# Autodesk Inventor assembly: Flywheel Axle Assembly v11
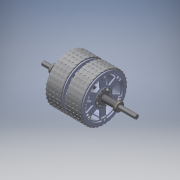
[picture p0: Inventor's stored thumbnail of the model, 180x180]
Saved by Autodesk Inventor 2018 (Build 220112000, 112)
## iProperties
Created: 2020-01-29
Part Number: Flywheel Axle Assembly v11
Document SubType Name: Assembly
Designer: s-2512711
Author: s-2512711
## Documents named in this file (10)
- \\studenthome\students\S-2512711\GitHub\2020CAD\New Gabriel Shooter\ACTUAL ASSEMBLY FILES\Flywheel Axle Assembly v11.iam
- \\studenthome\students\S-2512711\GitHub\2020CAD\New Gabriel Shooter\ACTUAL ASSEMBLY FILES\am-2986 FR8ZZ Hex Bearing v1.ipt
- \\studenthome\students\S-2512711\GitHub\2020CAD\New Gabriel Shooter\ACTUAL ASSEMBLY FILES\6_Traction_Tire_mounted_on_6_Traction_Wheel v1.iam
- \\studenthome\students\S-2512711\GitHub\2020CAD\New Gabriel Shooter\ACTUAL ASSEMBLY FILES\6_Traction_Tire_mounted_on_6_Traction_Wheel v1_1.iam
- \\studenthome\students\S-2512711\GitHub\2020CAD\New Gabriel Shooter\ACTUAL ASSEMBLY FILES\1_2_Hex_Bore_Aluminum_VersaHub_217-2592 v1.ipt
- \\studenthome\students\S-2512711\GitHub\2020CAD\New Gabriel Shooter\ACTUAL ASSEMBLY FILES\1_2_Acetal_Spacer_-_1_2_Hex_217-3261 v1.ipt
- \\studenthome\students\S-2512711\GitHub\2020CAD\New Gabriel Shooter\ACTUAL ASSEMBLY FILES\1_16_Acetal_Spacer_-_1_2_Hex_217-3257 v1.ipt
- \\studenthome\students\S-2512711\GitHub\2020CAD\New Gabriel Shooter\ACTUAL ASSEMBLY FILES\1_Acetal_Spacer_-_1_2_Hex_217-3263 v1.ipt
- \\studenthome\students\S-2512711\GitHub\2020CAD\New Gabriel Shooter\ACTUAL ASSEMBLY FILES\1_4_Acetal_Spacer_-_1_2_Hex_217-3259 v1.ipt
- \\studenthome\students\S-2512711\GitHub\2020CAD\New Gabriel Shooter\ACTUAL ASSEMBLY FILES\Flywheel Axle Assembly v11.ipt
## Components (18 placed, 8 different names)
1. am-2986 FR8ZZ Hex Bearing v1:1 — Mate:1, Mate:2, Flush:1
2. am-2986 FR8ZZ Hex Bearing v1:2 — Mate:30, Mate:31, Flush:8
3. 6_Traction_Tire_mounted_on_6_Traction_Wheel v1:1 [sub-assembly] — Mate:13, Mate:14, Mate:19, Mate:20
4. 6_Traction_Tire_mounted_on_6_Traction_Wheel v1:2 [sub-assembly] — Mate:24, Mate:25, Mate:26, Mate:29
5. 1_2_Hex_Bore_Aluminum_VersaHub_217-2592 v1:1 — Mate:11, Mate:12, Flush:6, Mate:13, Mate:14
6. 1_2_Hex_Bore_Aluminum_VersaHub_217-2592 v1:2 — Mate:17, Mate:18, Mate:19, Mate:20, Mate:23
7. 1_2_Hex_Bore_Aluminum_VersaHub_217-2592 v1:3 — Mate:15, Mate:16, Flush:7, Mate:24, Mate:25, Mate:26
8. 1_2_Hex_Bore_Aluminum_VersaHub_217-2592 v1:4 — Mate:27, Mate:28, Mate:29
9. 1_2_Acetal_Spacer_-_1_2_Hex_217-3261 v1:1 — Mate:21, Mate:22, Mate:23
10. 1_2_Acetal_Spacer_-_1_2_Hex_217-3261 v1:2 — Mate:7, Mate:8, Flush:4
11. 1_2_Acetal_Spacer_-_1_2_Hex_217-3261 v1:3 — Mate:36, Mate:37, Flush:11
12. 1_16_Acetal_Spacer_-_1_2_Hex_217-3257 v1:1 — Mate:32, Mate:33, Flush:9
13. 1_16_Acetal_Spacer_-_1_2_Hex_217-3257 v1:2 — Mate:3, Mate:4, Flush:2
14. 1_Acetal_Spacer_-_1_2_Hex_217-3263 v1:1 — Mate:38, Mate:39, Flush:12
15. 1_Acetal_Spacer_-_1_2_Hex_217-3263 v1:2 — Mate:9, Mate:10, Flush:5
16. 1_4_Acetal_Spacer_-_1_2_Hex_217-3259 v1:1 — Mate:5, Mate:6, Flush:3
17. 1_4_Acetal_Spacer_-_1_2_Hex_217-3259 v1:2 — Mate:34, Mate:35, Flush:10
18. Flywheel Axle Assembly v11 — Mate:1, Mate:2, Flush:1, Mate:3, Mate:4, Flush:2, Mate:5, Mate:6, Flush:3, Mate:7, Mate:8, Flush:4, Mate:9, Mate:10, Flush:5, Mate:11, Mate:12, Flush:6, Mate:15, Mate:16, Flush:7, Mate:17, Mate:18, Mate:21, Mate:22, Mate:27, Mate:28, Mate:30, Mate:31, Flush:8, Mate:32, Mate:33, Flush:9, Mate:34, Mate:35, Flush:10, Mate:36, Mate:37, Flush:11, Mate:38, Mate:39, Flush:12
## Relationships (51: Mate 39, Flush 12)
- Mate:1: am-2986 FR8ZZ Hex Bearing v1:1 ↔ Flywheel Axle Assembly v11
- Mate:2: am-2986 FR8ZZ Hex Bearing v1:1 ↔ Flywheel Axle Assembly v11
- Flush:1 (31.75 mm): am-2986 FR8ZZ Hex Bearing v1:1 ↔ Flywheel Axle Assembly v11
- Mate:3: 1_16_Acetal_Spacer_-_1_2_Hex_217-3257 v1:2 ↔ Flywheel Axle Assembly v11
- Mate:4: 1_16_Acetal_Spacer_-_1_2_Hex_217-3257 v1:2 ↔ Flywheel Axle Assembly v11
- Flush:2 (39.6875 mm): 1_16_Acetal_Spacer_-_1_2_Hex_217-3257 v1:2 ↔ Flywheel Axle Assembly v11
- Mate:5: 1_4_Acetal_Spacer_-_1_2_Hex_217-3259 v1:1 ↔ Flywheel Axle Assembly v11
- Mate:6: 1_4_Acetal_Spacer_-_1_2_Hex_217-3259 v1:1 ↔ Flywheel Axle Assembly v11
- Flush:3 (41.275 mm): 1_4_Acetal_Spacer_-_1_2_Hex_217-3259 v1:1 ↔ Flywheel Axle Assembly v11
- Mate:7: 1_2_Acetal_Spacer_-_1_2_Hex_217-3261 v1:2 ↔ Flywheel Axle Assembly v11
- Mate:8: 1_2_Acetal_Spacer_-_1_2_Hex_217-3261 v1:2 ↔ Flywheel Axle Assembly v11
- Flush:4 (47.625 mm): 1_2_Acetal_Spacer_-_1_2_Hex_217-3261 v1:2 ↔ Flywheel Axle Assembly v11
- Mate:9: 1_Acetal_Spacer_-_1_2_Hex_217-3263 v1:2 ↔ Flywheel Axle Assembly v11
- Mate:10: 1_Acetal_Spacer_-_1_2_Hex_217-3263 v1:2 ↔ Flywheel Axle Assembly v11
- Flush:5 (60.325 mm): 1_Acetal_Spacer_-_1_2_Hex_217-3263 v1:2 ↔ Flywheel Axle Assembly v11
- Mate:11: 1_2_Hex_Bore_Aluminum_VersaHub_217-2592 v1:1 ↔ Flywheel Axle Assembly v11
- Mate:12: 1_2_Hex_Bore_Aluminum_VersaHub_217-2592 v1:1 ↔ Flywheel Axle Assembly v11
- Flush:6 (85.725 mm): 1_2_Hex_Bore_Aluminum_VersaHub_217-2592 v1:1 ↔ Flywheel Axle Assembly v11
- Mate:13: 6_Traction_Tire_mounted_on_6_Traction_Wheel v1:1 ↔ 1_2_Hex_Bore_Aluminum_VersaHub_217-2592 v1:1
- Mate:14: 6_Traction_Tire_mounted_on_6_Traction_Wheel v1:1 ↔ 1_2_Hex_Bore_Aluminum_VersaHub_217-2592 v1:1
- Mate:15: 1_2_Hex_Bore_Aluminum_VersaHub_217-2592 v1:3 ↔ Flywheel Axle Assembly v11
- Mate:16: 1_2_Hex_Bore_Aluminum_VersaHub_217-2592 v1:3 ↔ Flywheel Axle Assembly v11
- Flush:7 (152.4 mm): 1_2_Hex_Bore_Aluminum_VersaHub_217-2592 v1:3 ↔ Flywheel Axle Assembly v11
- Mate:17: 1_2_Hex_Bore_Aluminum_VersaHub_217-2592 v1:2 ↔ Flywheel Axle Assembly v11
- Mate:18: 1_2_Hex_Bore_Aluminum_VersaHub_217-2592 v1:2 ↔ Flywheel Axle Assembly v11
- Mate:19: 6_Traction_Tire_mounted_on_6_Traction_Wheel v1:1 ↔ 1_2_Hex_Bore_Aluminum_VersaHub_217-2592 v1:2
- Mate:20: 6_Traction_Tire_mounted_on_6_Traction_Wheel v1:1 ↔ 1_2_Hex_Bore_Aluminum_VersaHub_217-2592 v1:2
- Mate:21: 1_2_Acetal_Spacer_-_1_2_Hex_217-3261 v1:1 ↔ Flywheel Axle Assembly v11
- Mate:22: 1_2_Acetal_Spacer_-_1_2_Hex_217-3261 v1:1 ↔ Flywheel Axle Assembly v11
- Mate:23: 1_2_Hex_Bore_Aluminum_VersaHub_217-2592 v1:2 ↔ 1_2_Acetal_Spacer_-_1_2_Hex_217-3261 v1:1
- Mate:24: 6_Traction_Tire_mounted_on_6_Traction_Wheel v1:2 ↔ 1_2_Hex_Bore_Aluminum_VersaHub_217-2592 v1:3
- Mate:25: 6_Traction_Tire_mounted_on_6_Traction_Wheel v1:2 ↔ 1_2_Hex_Bore_Aluminum_VersaHub_217-2592 v1:3
- Mate:26: 6_Traction_Tire_mounted_on_6_Traction_Wheel v1:2 ↔ 1_2_Hex_Bore_Aluminum_VersaHub_217-2592 v1:3
- Mate:27: 1_2_Hex_Bore_Aluminum_VersaHub_217-2592 v1:4 ↔ Flywheel Axle Assembly v11
- Mate:28: 1_2_Hex_Bore_Aluminum_VersaHub_217-2592 v1:4 ↔ Flywheel Axle Assembly v11
- Mate:29: 6_Traction_Tire_mounted_on_6_Traction_Wheel v1:2 ↔ 1_2_Hex_Bore_Aluminum_VersaHub_217-2592 v1:4
- Mate:30: am-2986 FR8ZZ Hex Bearing v1:2 ↔ Flywheel Axle Assembly v11
- Mate:31: am-2986 FR8ZZ Hex Bearing v1:2 ↔ Flywheel Axle Assembly v11
- Flush:8 (57.1602 mm): am-2986 FR8ZZ Hex Bearing v1:2 ↔ Flywheel Axle Assembly v11
- Mate:32: 1_16_Acetal_Spacer_-_1_2_Hex_217-3257 v1:1 ↔ Flywheel Axle Assembly v11
- Mate:33: 1_16_Acetal_Spacer_-_1_2_Hex_217-3257 v1:1 ↔ Flywheel Axle Assembly v11
- Flush:9 (65.0875 mm): 1_16_Acetal_Spacer_-_1_2_Hex_217-3257 v1:1 ↔ Flywheel Axle Assembly v11
- Mate:34: 1_4_Acetal_Spacer_-_1_2_Hex_217-3259 v1:2 ↔ Flywheel Axle Assembly v11
- Mate:35: 1_4_Acetal_Spacer_-_1_2_Hex_217-3259 v1:2 ↔ Flywheel Axle Assembly v11
- Flush:10 (66.675 mm): 1_4_Acetal_Spacer_-_1_2_Hex_217-3259 v1:2 ↔ Flywheel Axle Assembly v11
- Mate:36: 1_2_Acetal_Spacer_-_1_2_Hex_217-3261 v1:3 ↔ Flywheel Axle Assembly v11
- Mate:37: 1_2_Acetal_Spacer_-_1_2_Hex_217-3261 v1:3 ↔ Flywheel Axle Assembly v11
- Flush:11 (73.025 mm): 1_2_Acetal_Spacer_-_1_2_Hex_217-3261 v1:3 ↔ Flywheel Axle Assembly v11
- Mate:38: 1_Acetal_Spacer_-_1_2_Hex_217-3263 v1:1 ↔ Flywheel Axle Assembly v11
- Mate:39: 1_Acetal_Spacer_-_1_2_Hex_217-3263 v1:1 ↔ Flywheel Axle Assembly v11
- Flush:12 (85.725 mm): 1_Acetal_Spacer_-_1_2_Hex_217-3263 v1:1 ↔ Flywheel Axle Assembly v11
